# Autodesk Inventor assembly: HHPSJC5
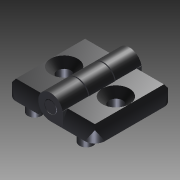
[picture p0: Inventor's stored thumbnail of the model, 180x180]
Saved by Autodesk Inventor 2015 SP1 (Build 190203100, 203)
## iProperties
Category: PARTsolutions
Company: MISUMI
Created: 2015-01-26
Part Number: HHPSJC5
Catalog Web Link: www.cadenas.de
Description: HHPSJC-Compact Resin Hinges
Vendor: MISUMI
Document SubType Name: Assembly
Designer: PARTuser1
Manufacturer: MISUMI
PSOL_IDENT_0: {\\10.0.0.236\data_v8\23d-libs\misumi\metric\39_accessories_for_al_extrusions\hhpsjc_asmtab.prj},164
PSOL_IDENT_1: {VTYP=3D},{STYP=ASSTAB},{NB=HHPSJC5},{LINA=HHPSJC5},{NN=HHPSJC},{DATE=17.11.2014 05:31:05},{GEOMDAT
PSOL_IDENT_2: E=11.03.2010},{VERSION=},{LINEID=10},{LINESUBID=-1},{WBVAR=ALT}  {NB=HHPSJC5},{LINA=HHPSJC5},{KT=DUM
PSOL_IDENT_3: MY},{PN=HHPSJC5},{TYPE=HHPSJC},{MATL=Nylon 6},{MATS=304 Stainless Steel},{NO=5},{ALKG=10},{ALN=98},{
PSOL_IDENT_4: MASS=12.5},{L=32},{W=36},{K=4},{P=24},{J=7.5},{S=21},{ND=5.5},{NC=11},{T=6},{TT=4},{E=10},{R=5.0},{A=
PSOL_IDENT_5: 5.5},{ALT=},{MATBOLT=},{MATNUT=316 Stainless Steel (or Equivalent)},{ND1=2.0},{LBOLT=8},{MSHFBS=5},{
PSOL_IDENT_6: PPATH=hhpsjc_amstpl.prj},{AB=FB5-8},{AN=HNTT5-5}
SUPPLIER: MISUMI
ARTICLENO: HHPSJC5
BOMINFO: HHPSJC5
CREATOR: CADENAS GmbH
Title: HHPSJC5
Author: Cadenas PARTsolutions
Comments: Compact Resin Hinges
## Documents named in this file (4)
- C:\Users\Jack\ownCloud\Projects\CoreXY\InventorModel\Hardware\Hinges\HingeHHPSJC5\HHPSJC5.iam
- C:\Users\Jack\ownCloud\Projects\CoreXY\InventorModel\Hardware\Hinges\HingeHHPSJC5\HHPSJC5_125_l.ipt
- C:\Users\Jack\ownCloud\Projects\CoreXY\InventorModel\Hardware\Hinges\HingeHHPSJC5\HHPSJC5_r.ipt
- C:\Users\Jack\ownCloud\Projects\CoreXY\InventorModel\Hardware\Hinges\HingeHHPSJC5\HHPSJC5_pin.ipt
## Components (3 placed, 3 different names)
1. HHPSJC5_125_l:1 — Mate:2
2. HHPSJC5_r:1 — Mate:1, Mate:2
3. HHPSJC5_pin:1 — Mate:1
## Relationships (2: Mate 2)
- Mate:1: HHPSJC5_r:1 ↔ HHPSJC5_pin:1
- Mate:2 (0.5 mm): HHPSJC5_125_l:1 ↔ HHPSJC5_r:1
